# Autodesk Inventor assembly: Arm
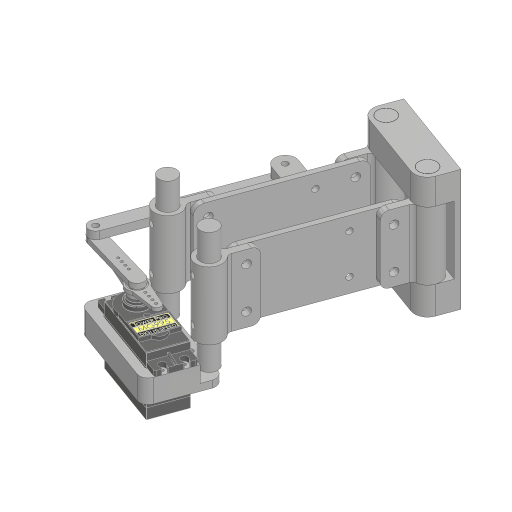
[picture p0: Inventor's stored thumbnail of the model, 512x512]
Saved by Autodesk Inventor 2024 (Build 280153000, 153)
## iProperties
Created: 2025-04-25
Part Number: Arm
Document SubType Name: Assembly
Designer: Binara
Author: Binara
## Documents named in this file (11)
- Z:\Robotics\Inventor\Auto Chair\Auto Chair\Arm.iam
- Z:\Robotics\Inventor\Auto Chair\Auto Chair\Bolt.ipt
- Z:\Robotics\Inventor\Auto Chair\Auto Chair\Axle Joint.ipt
- Z:\Robotics\Inventor\Auto Chair\Auto Chair\Top Arm Plate.ipt
- Z:\Robotics\Inventor\Auto Chair\Auto Chair\Mg995 v1.ipt
- Z:\Robotics\Inventor\Auto Chair\Auto Chair\Servo Mount.ipt
- Z:\Robotics\Inventor\Auto Chair\Auto Chair\MG995_Gear2 v1.ipt
- Z:\Robotics\Inventor\Auto Chair\Auto Chair\Servo Small Arm.ipt
- Z:\Robotics\Inventor\Auto Chair\Auto Chair\Arm Link.ipt
- Z:\Robotics\Inventor\Auto Chair\Auto Chair\Servo Long Arm.ipt
- Z:\Robotics\Inventor\Auto Chair\Auto Chair\Endpoint.ipt
## Components (17 placed, 10 different names)
1. Bolt:1
2. Axle Joint:1 — Rigid:4
3. Axle Joint:2 — Rigid:3
4. Bolt:2
5. Top Arm Plate:1 — Rigid:1, Rigid:4
6. Top Arm Plate:2 — Rigid:2, Rigid:3
7. Axle Joint:3 — Rigid:1
8. Axle Joint:4 — Rigid:2
9. Mg995 v1:1
10. Servo Mount:1
11. MG995_Gear2 v1:1
12. Servo Small Arm:1
13. Arm Link:1
14. Servo Long Arm:1
15. Bolt:5 — Rotational:1
16. Bolt:6 — Rotational:2
17. Endpoint:1 — Rotational:1, Rotational:2
## Relationships (6: WeldJoint 4, RevoluteJoint 2)
- Rotational:1 [RevoluteJoint]: Bolt:5 ↔ Endpoint:1
- Rotational:2 [RevoluteJoint]: Bolt:6 ↔ Endpoint:1
- Rigid:1 [WeldJoint]: Top Arm Plate:1 ↔ Axle Joint:3
- Rigid:2 [WeldJoint]: Top Arm Plate:2 ↔ Axle Joint:4
- Rigid:3 [WeldJoint]: Axle Joint:2 ↔ Top Arm Plate:2
- Rigid:4 [WeldJoint]: Axle Joint:1 ↔ Top Arm Plate:1
